# Autodesk Inventor assembly: BOWDEN DRIVE
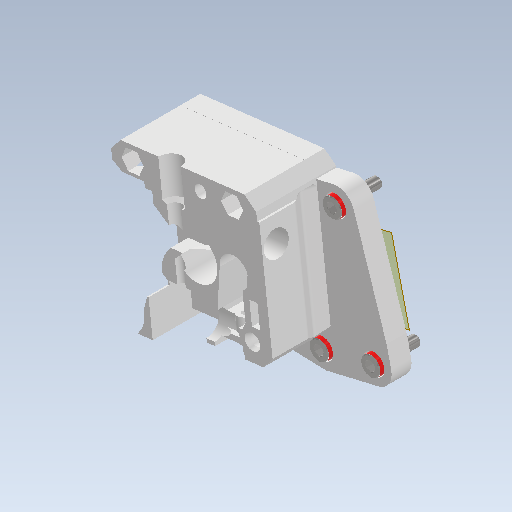
[picture p0: Inventor's stored thumbnail of the model, 512x512]
Saved by Autodesk Inventor 2020.3 (Build 243373010, 373A)
## iProperties
Created: 2019-11-12
Part Number: BOWDEN DRIVE
Document SubType Name: Assembly
Designer: pepd9
Author: pepd9
## Documents named in this file (4)
- D:\Designs\MK3PRO P1\BOWDEN DRIVE\BOWDEN DRIVE.iam
- D:\Designs\MK3PRO P1\BOWDEN DRIVE\BOWDEN MOUNT.ipt
- D:\Designs\MK3PRO P1\BOWDEN DRIVE\extruder-body.ipt
- D:\Designs\MK3PRO P1\COMPONENTS\SHCS_M3_8.ipt
## Components (5 placed, 3 different names)
1. BOWDEN MOUNT:1 — Mate:1, Mate:6, Mate:7, Mate:8, Mate:9, Mate:10, Mate:11, Mate:14, Mate:15
2. extruder-body:1 — Mate:1, Mate:14, Mate:15
3. SHCS_M3_8:2 — Mate:6, Mate:9
4. SHCS_M3_8:3 — Mate:7, Mate:8
5. SHCS_M3_8:4 — Mate:10, Mate:11
## Relationships (9: Mate 9)
- Mate:1: BOWDEN MOUNT:1 ↔ extruder-body:1
- Mate:6: BOWDEN MOUNT:1 ↔ SHCS_M3_8:2
- Mate:7: BOWDEN MOUNT:1 ↔ SHCS_M3_8:3
- Mate:8: BOWDEN MOUNT:1 ↔ SHCS_M3_8:3
- Mate:9: BOWDEN MOUNT:1 ↔ SHCS_M3_8:2
- Mate:10: BOWDEN MOUNT:1 ↔ SHCS_M3_8:4
- Mate:11: BOWDEN MOUNT:1 ↔ SHCS_M3_8:4
- Mate:14: BOWDEN MOUNT:1 ↔ extruder-body:1
- Mate:15: BOWDEN MOUNT:1 ↔ extruder-body:1
